# Autodesk Inventor assembly: enc-BackPanel MitteRechts - Assembly
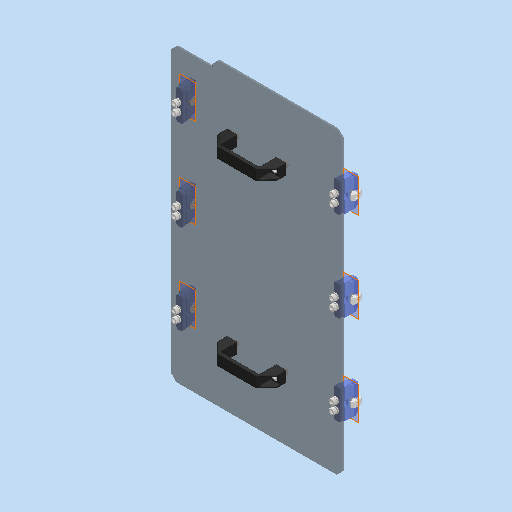
[picture p0: Inventor's stored thumbnail of the model, 512x512]
Saved by Autodesk Inventor 2023.2 (Build 272271000, 271)
## iProperties
Created: 2023-12-04
Part Number: enc-BackPanel MitteRechts - Assembly
Document SubType Name: Assembly
Designer: Nils Bade
Author: Nils Bade
## Documents named in this file (6)
- C:\Users\nilsb\Documents\Inventor\Projektarbeit-Bade\Enclosure\enc-BackPanel MitteRechts - Assembly.iam
- C:\Users\nilsb\Documents\Inventor\Projektarbeit-Bade\Enclosure\V-Slot Door Handle v1.ipt
- C:\Users\nilsb\Documents\Inventor\Projektarbeit-Bade\Schrauben\Cap Head Screw M6x16 - DIN912.ipt
- C:\Users\nilsb\Documents\Inventor\Projektarbeit-Bade\RatRig_Standards\Hex Locking Nut - M6 v2.ipt
- C:\Users\nilsb\Documents\Inventor\Projektarbeit-Bade\Enclosure\Magnet PanelFrame 90deg connected.iam
- C:\Users\nilsb\Documents\Inventor\Projektarbeit-Bade\Enclosure\enc-BackPanel Mitte.ipt
## Components (17 placed, 5 different names)
1. V-Slot Door Handle v1:1 — Passend:12, Passend:13, Passend:21, Passend:22
2. V-Slot Door Handle v1:2 — Passend:17, Passend:18, Passend:19, Passend:20
3. Cap Head Screw M6x16 - DIN912:1 — Passend:3, Passend:12, Passend:22
4. Cap Head Screw M6x16 - DIN912:2 — Passend:4, Passend:13, Passend:21
5. Cap Head Screw M6x16 - DIN912:3 — Passend:2, Passend:18, Passend:19
6. Cap Head Screw M6x16 - DIN912:4 — Passend:1, Passend:17, Passend:20
7. Hex Locking Nut - M6 v2:1 — Passend:3
8. Hex Locking Nut - M6 v2:2 — Passend:4
9. Hex Locking Nut - M6 v2:3 — Passend:2
10. Hex Locking Nut - M6 v2:4 — Passend:1
11. Magnet PanelFrame 90deg connected:1 [sub-assembly]
12. Magnet PanelFrame 90deg connected:2 [sub-assembly]
13. Magnet PanelFrame 90deg connected:3 [sub-assembly]
14. Magnet PanelFrame 90deg connected:4 [sub-assembly]
15. Magnet PanelFrame 90deg connected:5 [sub-assembly]
16. Magnet PanelFrame 90deg connected:6 [sub-assembly]
17. enc-BackPanel Mitte:1
## Relationships (15: Mate 15)
- Passend:1 [Mate]: Cap Head Screw M6x16 - DIN912:4 ↔ Hex Locking Nut - M6 v2:4
- Passend:2 [Mate]: Cap Head Screw M6x16 - DIN912:3 ↔ Hex Locking Nut - M6 v2:3
- Passend:3 [Mate]: Cap Head Screw M6x16 - DIN912:1 ↔ Hex Locking Nut - M6 v2:1
- Passend:4 [Mate]: Cap Head Screw M6x16 - DIN912:2 ↔ Hex Locking Nut - M6 v2:2
- Passend:12 [Mate]: V-Slot Door Handle v1:1 ↔ Cap Head Screw M6x16 - DIN912:1
- Passend:13 [Mate]: V-Slot Door Handle v1:1 ↔ Cap Head Screw M6x16 - DIN912:2
- Passend:17 [Mate]: V-Slot Door Handle v1:2 ↔ Cap Head Screw M6x16 - DIN912:4
- Passend:18 [Mate]: V-Slot Door Handle v1:2 ↔ Cap Head Screw M6x16 - DIN912:3
- Passend:19 [Mate]: V-Slot Door Handle v1:2 ↔ Cap Head Screw M6x16 - DIN912:3
- Passend:20 [Mate]: V-Slot Door Handle v1:2 ↔ Cap Head Screw M6x16 - DIN912:4
- Passend:21 [Mate]: V-Slot Door Handle v1:1 ↔ Cap Head Screw M6x16 - DIN912:2
- Passend:22 [Mate]: V-Slot Door Handle v1:1 ↔ Cap Head Screw M6x16 - DIN912:1
- [Mate]: Magnet PanelFrame 90deg connected:4 ↔ enc-BackPanel Mitte:1
- [Mate]: Magnet PanelFrame 90deg connected:3 ↔ enc-BackPanel Mitte:1
- [Mate]: Magnet PanelFrame 90deg connected:3 ↔ enc-BackPanel Mitte:1
